# Autodesk Inventor assembly: Montagem
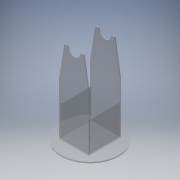
[picture p0: Inventor's stored thumbnail of the model, 180x180]
Saved by Autodesk Inventor 2016 (Build 200138000, 138)
## iProperties
Created: 2017-04-03
Part Number: Montagem
Document SubType Name: Assembly
Designer: Marcelo
Author: Marcelo
## Documents named in this file (5)
- D:\Users\Marcelo\Documents\GitHub\telescopiocaseiro\Hardware\PT-001\Montagem.iam
- D:\Users\Marcelo\Documents\GitHub\telescopiocaseiro\Hardware\PT-001\DiscoAzimute.ipt
- D:\Users\Marcelo\Documents\GitHub\telescopiocaseiro\Hardware\PT-001\Afastador.ipt
- D:\Users\Marcelo\Documents\GitHub\telescopiocaseiro\Hardware\PT-001\Suporte.ipt
- D:\Users\Marcelo\Documents\GitHub\telescopiocaseiro\Hardware\PT-001\Base.ipt
## Components (6 placed, 4 different names)
1. DiscoAzimute:1 — Mate:8, Mate:9
2. Suporte:1 — Mate:4, Flush:7, Flush:8, Flush:10, Flush:11, Flush:12, Mate:7
3. Suporte:2 — Flush:5, Mate:5, Flush:6, Flush:9, Mate:6
4. Afastador:2 — Mate:4, Flush:5, Mate:5, Flush:6, Flush:7, Flush:8, Flush:9
5. Afastador:3 — Mate:6, Flush:10, Flush:11, Flush:13
6. Base:1 — Flush:12, Flush:13, Mate:7, Mate:8, Mate:9
## Relationships (15: Flush 9, Mate 6)
- Mate:4: Suporte:1 ↔ Afastador:2
- Flush:5: Suporte:2 ↔ Afastador:2
- Mate:5: Suporte:2 ↔ Afastador:2
- Flush:6: Suporte:2 ↔ Afastador:2
- Flush:7: Suporte:1 ↔ Afastador:2
- Flush:8: Suporte:1 ↔ Afastador:2
- Flush:9: Suporte:2 ↔ Afastador:2
- Mate:6: Suporte:2 ↔ Afastador:3
- Flush:10: Suporte:1 ↔ Afastador:3
- Flush:11: Suporte:1 ↔ Afastador:3
- Flush:12: Suporte:1 ↔ Base:1
- Flush:13: Afastador:3 ↔ Base:1
- Mate:7: Suporte:1 ↔ Base:1
- Mate:8: DiscoAzimute:1 ↔ Base:1
- Mate:9: DiscoAzimute:1 ↔ Base:1
